# Autodesk Inventor assembly: __VK_WT_ZSB
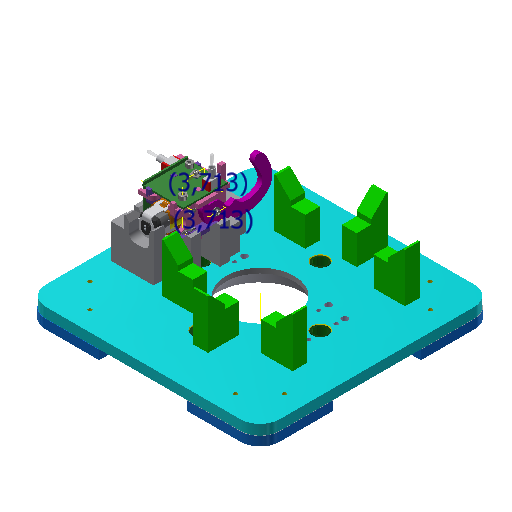
[picture p0: Inventor's stored thumbnail of the model, 512x512]
Saved by Autodesk Inventor 2025.1 (Build 291241000, 241)
## iProperties
Created: 2023-11-18
Part Number: __VK_WT_ZSB
Material: Generisch
Document SubType Name: Assembly
Designer: RP
Author: RP
## Documents named in this file (3)
- C:\Users\Erik\Erik\Hochschule\3. Semester\CAD\CAD-Paspa\Useless Box\_Verkettung\__VK_WT_beladen.iam
- C:\Users\Erik\Erik\Hochschule\3. Semester\CAD\CAD-Paspa\Useless Box\_Verkettung\__VK_WT.iam
- C:\Users\Erik\Erik\Hochschule\3. Semester\CAD\CAD-Paspa\Useless Box\_Useless_Box\Antriebseinheit_ZSB.iam
## Components (3 placed, 2 different names)
1. __VK_WT:1 [sub-assembly] — Fluchtend:16, Fluchtend:17, Fluchtend:18
2. Antriebseinheit_ZSB:1 [sub-assembly]
3. Antriebseinheit_ZSB:2 [sub-assembly]
## Relationships (16: Mate 12, Flush 4)
- [Flush]: __VK_WT:1
- [Mate]: __VK_WT:1
- [Mate] (20.3 mm): __VK_WT:1
- Fluchtend:16 [Flush]: __VK_WT:1
- Fluchtend:17 [Flush]: __VK_WT:1
- Fluchtend:18 [Flush]: __VK_WT:1
- [Mate]: __VK_WT:1 ↔ Antriebseinheit_ZSB:1
- [Mate]: __VK_WT:1 ↔ Antriebseinheit_ZSB:1
- [Mate]: __VK_WT:1 ↔ Antriebseinheit_ZSB:1
- [Mate]: __VK_WT:1 ↔ Antriebseinheit_ZSB:2
- [Mate]: __VK_WT:1 ↔ Antriebseinheit_ZSB:2
- [Mate]: __VK_WT:1 ↔ Antriebseinheit_ZSB:2
- [Mate]: __VK_WT:1 ↔ Antriebseinheit_ZSB:1
- [Mate]: __VK_WT:1 ↔ Antriebseinheit_ZSB:1
- [Mate]: __VK_WT:1 ↔ Antriebseinheit_ZSB:1
- [Mate]: __VK_WT:1 ↔ Antriebseinheit_ZSB:1
